# Autodesk Inventor assembly: Foot_MIR
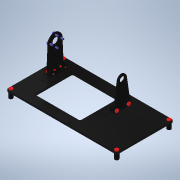
[picture p0: Inventor's stored thumbnail of the model, 180x180]
Saved by Autodesk Inventor 2022 (Build 260153000, 153)
## iProperties
Created: 2022-06-04
Part Number: Foot_MIR
Document SubType Name: Assembly
Designer: Masato Kubotera
Author: Masato Kubotera
## Documents named in this file (9)
- C:\Users\MasatoKubotera\Documents\Inventor\SUSTAINA-OP\LowerBody\Foot\Foot_MIR.iam
- C:\Users\MasatoKubotera\Documents\Inventor\SUSTAINA-OP\LowerBody\Foot\Sole_frame.ipt
- C:\Users\MasatoKubotera\Documents\Inventor\SUSTAINA-OP\LowerBody\Foot\Foot_front_frame.ipt
- C:\Users\MasatoKubotera\Documents\Inventor\SUSTAINA-OP\LowerBody\Foot\Foot_back_frame.ipt
- C:\Users\MasatoKubotera\Documents\Inventor\SUSTAINA-OP\LowerBody\Foot\Foot_root_block.ipt
- C:\Users\MasatoKubotera\Documents\Inventor\SUSTAINA-OP\ReadyMade\Spacer\ASL-309BE.ipt
- C:\Users\MasatoKubotera\Documents\Inventor\SUSTAINA-OP\ReadyMade\Screw\M3-10.ipt
- C:\Users\MasatoKubotera\Documents\Inventor\SUSTAINA-OP\ReadyMade\Screw\M3-8.ipt
- C:\Users\MasatoKubotera\Documents\Inventor\SUSTAINA-OP\ReadyMade\Screw\M2_6-6.ipt
## Components (25 placed, 8 different names)
1. Sole_frame:1 — 挿入:2, 挿入:1, 挿入:4, 挿入:3, 挿入:13, 挿入:14, 挿入:15, 挿入:16, 挿入:21, 挿入:22, 挿入:23, 挿入:24, 挿入:25, 挿入:26, 挿入:27, 挿入:28
2. Foot_front_frame:1 — メイト:2, メイト:1, 挿入:6, 挿入:5, 挿入:31, 挿入:32
3. Foot_back_frame:1 — 挿入:8, 挿入:7, 挿入:17, 挿入:18, 挿入:19, 挿入:20, 挿入:29, 挿入:30
4. Foot_root_block:1 — 挿入:6, 挿入:5, 挿入:2, 挿入:1
5. Foot_root_block:2 — 挿入:8, 挿入:7, 挿入:4, 挿入:3
6. ASL-309BE:1 — メイト:3, 挿入:21, 角度:1
7. ASL-309BE:2 — 挿入:22, 角度:2
8. ASL-309BE:3 — 挿入:23, 角度:3
9. ASL-309BE:4 — 挿入:24, 角度:4
10. M3-10:1 — 挿入:25
11. M3-10:2 — 挿入:26
12. M3-10:3 — 挿入:27
13. M3-10:4 — 挿入:28
14. M3-8:1 — 挿入:13
15. M3-8:2 — 挿入:14
16. M3-8:3 — 挿入:15
17. M3-8:4 — 挿入:16
18. M3-8:5 — 挿入:32
19. M3-8:6 — 挿入:31
20. M3-8:7 — 挿入:30
21. M3-8:8 — 挿入:29
22. M2_6-6:1 — 挿入:17
23. M2_6-6:2 — 挿入:18
24. M2_6-6:3 — 挿入:19
25. M2_6-6:4 — 挿入:20
## Relationships (35: Insert 28, Angle 4, Mate 3)
- メイト:2 [Mate]: Foot_front_frame:1
- メイト:1 [Mate]: Foot_front_frame:1
- 挿入:6 [Insert]: Foot_front_frame:1 ↔ Foot_root_block:1
- 挿入:5 [Insert]: Foot_front_frame:1 ↔ Foot_root_block:1
- 挿入:2 [Insert]: Sole_frame:1 ↔ Foot_root_block:1
- 挿入:1 [Insert]: Sole_frame:1 ↔ Foot_root_block:1
- 挿入:8 [Insert]: Foot_back_frame:1 ↔ Foot_root_block:2
- 挿入:7 [Insert]: Foot_back_frame:1 ↔ Foot_root_block:2
- 挿入:4 [Insert]: Sole_frame:1 ↔ Foot_root_block:2
- 挿入:3 [Insert]: Sole_frame:1 ↔ Foot_root_block:2
- 挿入:13 [Insert]: Sole_frame:1 ↔ M3-8:1
- 挿入:14 [Insert]: Sole_frame:1 ↔ M3-8:2
- 挿入:15 [Insert]: Sole_frame:1 ↔ M3-8:3
- 挿入:16 [Insert]: Sole_frame:1 ↔ M3-8:4
- 挿入:17 [Insert]: Foot_back_frame:1 ↔ M2_6-6:1
- 挿入:18 [Insert]: Foot_back_frame:1 ↔ M2_6-6:2
- 挿入:19 [Insert]: Foot_back_frame:1 ↔ M2_6-6:3
- 挿入:20 [Insert]: Foot_back_frame:1 ↔ M2_6-6:4
- メイト:3 [Mate]: ASL-309BE:1
- 挿入:21 [Insert]: Sole_frame:1 ↔ ASL-309BE:1
- 挿入:22 [Insert]: Sole_frame:1 ↔ ASL-309BE:2
- 挿入:23 [Insert]: Sole_frame:1 ↔ ASL-309BE:3
- 挿入:24 [Insert]: Sole_frame:1 ↔ ASL-309BE:4
- 挿入:25 [Insert]: Sole_frame:1 ↔ M3-10:1
- 挿入:26 [Insert]: Sole_frame:1 ↔ M3-10:2
- 挿入:27 [Insert]: Sole_frame:1 ↔ M3-10:3
- 挿入:28 [Insert]: Sole_frame:1 ↔ M3-10:4
- 挿入:29 [Insert]: Foot_back_frame:1 ↔ M3-8:8
- 挿入:30 [Insert]: Foot_back_frame:1 ↔ M3-8:7
- 挿入:31 [Insert]: Foot_front_frame:1 ↔ M3-8:6
- 挿入:32 [Insert]: Foot_front_frame:1 ↔ M3-8:5
- 角度:1 [Angle] (0 deg): ASL-309BE:1
- 角度:2 [Angle] (0 deg): ASL-309BE:2
- 角度:3 [Angle] (0 deg): ASL-309BE:3
- 角度:4 [Angle] (0 deg): ASL-309BE:4
